# Autodesk Inventor assembly: !Crossbrace
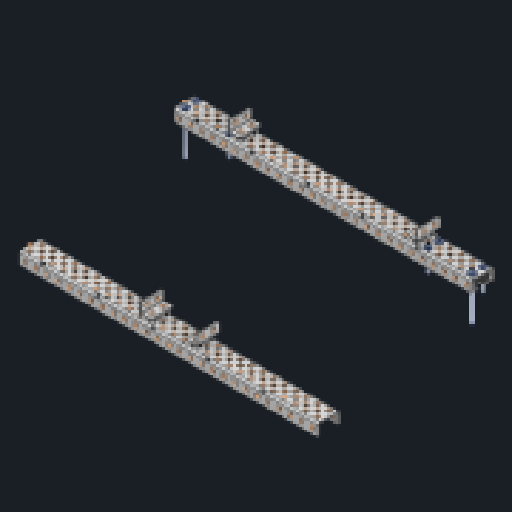
[picture p0: Inventor's stored thumbnail of the model, 512x512]
Saved by Autodesk Inventor 2025 (Build 290162000, 162)
## iProperties
Created: 2024-12-18
Part Number: !Crossbrace
Document SubType Name: Assembly
Designer: avere
Author: avere
## Documents named in this file (10)
- D:\VEX\High Stakes\CAD\V4\Chassis\Crossbrace\!Crossbrace.iam
- D:\VEX\High Stakes\CAD\ROBOPROS-CAD-Inventor\Structure\C Channel\Aluminum 1x2x1\Alu C 1x2x1x27.ipt
- D:\VEX\High Stakes\CAD\ROBOPROS-CAD-Inventor\Motion\Spacers\Spacer Nylon .375 OD\NSpacer .375 OD x .500.ipt
- D:\VEX\High Stakes\CAD\ROBOPROS-CAD-Inventor\Motion\Spacers\Spacer Nylon .375 OD.ipt
- D:\VEX\High Stakes\CAD\ROBOPROS-CAD-Inventor\Structure\Hardware\Screw Shoulder Robosource\SScrew Shoulder Smooth 2.000 x .04.ipt
- D:\VEX\High Stakes\CAD\ROBOPROS-CAD-Inventor\Structure\Hardware\Screw Shoulder Robosource.ipt
- D:\VEX\High Stakes\CAD\ROBOPROS-CAD-Inventor\Structure\Hardware\Screw Steel - Star\SScrew Star Smooth 1.000.ipt
- D:\VEX\High Stakes\CAD\ROBOPROS-CAD-Inventor\Structure\Hardware\Screw Steel - Star.ipt
- D:\VEX\High Stakes\CAD\ROBOPROS-CAD-Inventor\Modified Parts\Bearing Flat Low Profile 2-Hole.ipt
- D:\VEX\High Stakes\CAD\ROBOPROS-CAD-Inventor\Structure\Angle\Aluminum 1x1\Alu Angle 1x1x2.ipt
## Components (26 placed, 6 different names)
1. Alu C 1x2x1x27:1 — Mate:1, Flush:1, Flush:2, Mate:2, Mate:3, Flush:3, Insert:20, Mate:4, Insert:32, Mate:16
2. Alu C 1x2x1x27:2 — Mate:2, Mate:3, Flush:3, Insert:1, Insert:2, Insert:3, Insert:4, Insert:5, Insert:6, Insert:7, Insert:8, Insert:9, Insert:11, Insert:14, Insert:15, Insert:16, Insert:17, Insert:18, Insert:19, Insert:27, Mate:11, Insert:29, Mate:13
3. NSpacer .375 OD x .500:1 — Insert:4
4. NSpacer .375 OD x .500:2 — Insert:3
5. NSpacer .375 OD x .500:3 — Insert:2
6. NSpacer .375 OD x .500:4 — Insert:1
7. NSpacer .375 OD x .500:5 — Insert:6
8. NSpacer .375 OD x .500:6 — Insert:5
9. NSpacer .375 OD x .500:7 — Insert:8
10. NSpacer .375 OD x .500:8 — Insert:7
11. SScrew Shoulder Smooth 2.000 x .04:2 — Insert:9
12. SScrew Shoulder Smooth 2.000 x .04:4 — Insert:11
13. SScrew Star Smooth 1.000:1 — Insert:15
14. SScrew Star Smooth 1.000:2 — Insert:14
15. SScrew Star Smooth 1.000:3 — Insert:16
16. SScrew Star Smooth 1.000:4 — Insert:17
17. SScrew Star Smooth 1.000:5 — Insert:18
18. SScrew Star Smooth 1.000:6 — Insert:19
19. Bearing Flat Low Profile 2-Hole:1 — Insert:31, Mate:15, Insert:32, Mate:16
20. Bearing Flat Low Profile 2-Hole:2 — Insert:20, Mate:4, Insert:30, Mate:14
21. Alu Angle 1x1x2:1 — Insert:30, Mate:14
22. Alu Angle 1x1x2:2 — Insert:31, Mate:15
23. Bearing Flat Low Profile 2-Hole:3 — Insert:27
24. Alu Angle 1x1x2:3 — Mate:11
25. Bearing Flat Low Profile 2-Hole:4 — Insert:29
26. Alu Angle 1x1x2:4 — Mate:13
## Relationships (38: Insert 24, Mate 11, Flush 3)
- Mate:1 (76.2 mm): Alu C 1x2x1x27:1
- Flush:1 (-171.45 mm): Alu C 1x2x1x27:1
- Flush:2 (-17.4625 mm): Alu C 1x2x1x27:1
- Mate:2 (39.6875 mm): Alu C 1x2x1x27:1 ↔ Alu C 1x2x1x27:2
- Mate:3 (152.4 mm): Alu C 1x2x1x27:1 ↔ Alu C 1x2x1x27:2
- Flush:3: Alu C 1x2x1x27:1 ↔ Alu C 1x2x1x27:2
- Insert:1: Alu C 1x2x1x27:2 ↔ NSpacer .375 OD x .500:4
- Insert:2: Alu C 1x2x1x27:2 ↔ NSpacer .375 OD x .500:3
- Insert:3: Alu C 1x2x1x27:2 ↔ NSpacer .375 OD x .500:2
- Insert:4: Alu C 1x2x1x27:2 ↔ NSpacer .375 OD x .500:1
- Insert:5: Alu C 1x2x1x27:2 ↔ NSpacer .375 OD x .500:6
- Insert:6: Alu C 1x2x1x27:2 ↔ NSpacer .375 OD x .500:5
- Insert:7: Alu C 1x2x1x27:2 ↔ NSpacer .375 OD x .500:8
- Insert:8: Alu C 1x2x1x27:2 ↔ NSpacer .375 OD x .500:7
- Insert:9: Alu C 1x2x1x27:2 ↔ SScrew Shoulder Smooth 2.000 x .04:2
- Insert:11: Alu C 1x2x1x27:2 ↔ SScrew Shoulder Smooth 2.000 x .04:4
- Insert:14: Alu C 1x2x1x27:2 ↔ SScrew Star Smooth 1.000:2
- Insert:15: Alu C 1x2x1x27:2 ↔ SScrew Star Smooth 1.000:1
- Insert:16: Alu C 1x2x1x27:2 ↔ SScrew Star Smooth 1.000:3
- Insert:17: Alu C 1x2x1x27:2 ↔ SScrew Star Smooth 1.000:4
- Insert:18: Alu C 1x2x1x27:2 ↔ SScrew Star Smooth 1.000:5
- Insert:19: Alu C 1x2x1x27:2 ↔ SScrew Star Smooth 1.000:6
- Insert:20: Alu C 1x2x1x27:1 ↔ Bearing Flat Low Profile 2-Hole:2
- Mate:4: Alu C 1x2x1x27:1 ↔ Bearing Flat Low Profile 2-Hole:2
- [Insert] (1.27 mm): Bearing Flat Low Profile 2-Hole:3 ↔ Alu Angle 1x1x2:3
- [Mate]: Bearing Flat Low Profile 2-Hole:3 ↔ Alu Angle 1x1x2:3
- Insert:27: Alu C 1x2x1x27:2 ↔ Bearing Flat Low Profile 2-Hole:3
- Mate:11: Alu C 1x2x1x27:2 ↔ Alu Angle 1x1x2:3
- [Insert] (1.27 mm): Bearing Flat Low Profile 2-Hole:4 ↔ Alu Angle 1x1x2:4
- [Mate]: Bearing Flat Low Profile 2-Hole:4 ↔ Alu Angle 1x1x2:4
- Insert:29: Alu C 1x2x1x27:2 ↔ Bearing Flat Low Profile 2-Hole:4
- Mate:13: Alu C 1x2x1x27:2 ↔ Alu Angle 1x1x2:4
- Insert:30 (1.27 mm): Bearing Flat Low Profile 2-Hole:2 ↔ Alu Angle 1x1x2:1
- Mate:14: Bearing Flat Low Profile 2-Hole:2 ↔ Alu Angle 1x1x2:1
- Insert:31 (1.27 mm): Bearing Flat Low Profile 2-Hole:1 ↔ Alu Angle 1x1x2:2
- Mate:15: Bearing Flat Low Profile 2-Hole:1 ↔ Alu Angle 1x1x2:2
- Insert:32: Alu C 1x2x1x27:1 ↔ Bearing Flat Low Profile 2-Hole:1
- Mate:16: Alu C 1x2x1x27:1 ↔ Bearing Flat Low Profile 2-Hole:1
## Named parameters: d38_d36 = 1.27 mm, d39_d37 = 0 mm, d42_d38_d36 = 1.27 mm, d43_d39_d37 = 0 mm
